# Autodesk Inventor assembly: Сборка сортировщика
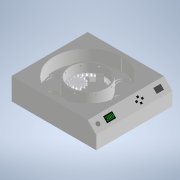
[picture p0: Inventor's stored thumbnail of the model, 180x180]
Saved by Autodesk Inventor 2022 (Build 260153000, 153)
## iProperties
Created: 2022-06-19
Part Number: Сборка сортировщика
Document SubType Name: Assembly
Designer: Admin
Author: Admin
## Documents named in this file (16)
- C:\Users\aleks\OneDrive\Рабочий стол\Проект хроматографического сборщика\Сборка сортировщика.iam
- C:\Users\aleks\OneDrive\Рабочий стол\Проект хроматографического сборщика\Барабан.ipt
- C:\Users\aleks\OneDrive\Рабочий стол\Проект хроматографического сборщика\Корпус.ipt
- C:\Users\aleks\OneDrive\Рабочий стол\Проект хроматографического сборщика\короб для подшипника.ipt
- C:\Users\aleks\OneDrive\Рабочий стол\Проект хроматографического сборщика\штырёк.ipt
- C:\Users\aleks\OneDrive\Рабочий стол\Проект хроматографического сборщика\Подшипник.ipt
- C:\Users\aleks\OneDrive\Рабочий стол\Проект хроматографического сборщика\Шаговик.ipt
- C:\Users\aleks\OneDrive\Рабочий стол\Старый сортировщик\Хромотаграфический сборщик модель\Детали\Вал.ipt
- C:\Users\aleks\OneDrive\Рабочий стол\Проект хроматографического сборщика\Healical Gear (12R@30.00 m=3.0).ipt
- C:\Users\aleks\OneDrive\Рабочий стол\Проект хроматографического сборщика\Healical Gear (32R@30.00 m=3.0).ipt
- C:\Users\aleks\OneDrive\Рабочий стол\Проект хроматографического сборщика\Держатель лазера.ipt
- C:\Users\aleks\OneDrive\Рабочий стол\Проект хроматографического сборщика\Лазер.ipt
- C:\Users\aleks\OneDrive\Рабочий стол\Проект хроматографического сборщика\Дисплей.ipt
- C:\Users\aleks\OneDrive\Рабочий стол\Проект хроматографического сборщика\Кнопки на плате.iam
- C:\Users\aleks\OneDrive\Рабочий стол\Проект хроматографического сборщика\Кнопка.ipt
- C:\Users\aleks\OneDrive\Рабочий стол\Проект хроматографического сборщика\Измеритель заряда.ipt
## Components (24 placed, 15 different names)
1. Барабан:1 — Заподлицо:1, Заподлицо:2, Заподлицо:3, Заподлицо:4, Совмещение:1, Совмещение:2, Совмещение:3, Совмещение:4, Совмещение:5, Совмещение:6, Совмещение:7, Совмещение:8, Заподлицо:5, Совмещение:9, Совмещение:15, ЗубчПер:2
2. Корпус:1 — Заподлицо:5, Совмещение:9, Совмещение:10, Совмещение:11, Совмещение:12, Совмещение:16, Совмещение:17, Совмещение:18, Совмещение:20, Совмещение:21, Заподлицо:8, Совмещение:22, Совмещение:23, Заподлицо:9, Совмещение:24, Совмещение:25, Совмещение:26, Совмещение:27, Совмещение:28
3. короб для подшипника:1 — Жесткий:2, Заподлицо:4, Совмещение:7, Совмещение:8
4. короб для подшипника:2 — Жесткий:1, Заподлицо:1, Совмещение:1, Совмещение:2
5. короб для подшипника:3 — Жесткий:3, Заподлицо:2, Совмещение:5, Совмещение:6
6. короб для подшипника:4 — Жесткий:4, Заподлицо:3, Совмещение:3, Совмещение:4
7. штырёк:2 — С поворотом:1, Жесткий:1
8. штырёк:3 — С поворотом:3, Жесткий:3
9. штырёк:4 — С поворотом:4, Жесткий:4
10. штырёк:5 — С поворотом:2, Жесткий:2
11. Подшипник:1 — С поворотом:1
12. Подшипник:2 — С поворотом:2
13. Подшипник:3 — С поворотом:3
14. Подшипник:4 — С поворотом:4
15. Шаговик:1 — Совмещение:10, Совмещение:11, Совмещение:12, Совмещение:13, Совмещение:14
16. Вал:1 — Совмещение:13, Совмещение:14, С поворотом:5
17. Healical Gear (12R@30.00 m=3.0):1 — С поворотом:5, Заподлицо:6, ЗубчПер:1
18. Healical Gear (32R@30.00 m=3.0):1 — Совмещение:15, Заподлицо:6, ЗубчПер:1, ЗубчПер:2
19. Держатель лазера:1 — Совмещение:16, Совмещение:17, Совмещение:18, Совмещение:19, Заподлицо:7
20. Лазер:1 — Совмещение:19, Заподлицо:7
21. Дисплей:1 — Заподлицо:9, Совмещение:24, Совмещение:25
22. Кнопки на плате:1 [sub-assembly] — Совмещение:26, Совмещение:27, Совмещение:28
23. Кнопка:1 — Совмещение:20, Совмещение:21
24. Измеритель заряда:1 — Заподлицо:8, Совмещение:22, Совмещение:23
## Relationships (48: Mate 28, Flush 9, RevoluteJoint 5, WeldJoint 4, RelateRotation 2)
- С поворотом:1 [RevoluteJoint]: штырёк:2 ↔ Подшипник:1
- С поворотом:2 [RevoluteJoint]: штырёк:5 ↔ Подшипник:2
- С поворотом:3 [RevoluteJoint]: штырёк:3 ↔ Подшипник:3
- С поворотом:4 [RevoluteJoint]: штырёк:4 ↔ Подшипник:4
- Жесткий:1 [WeldJoint]: короб для подшипника:2 ↔ штырёк:2
- Жесткий:2 [WeldJoint]: короб для подшипника:1 ↔ штырёк:5
- Жесткий:3 [WeldJoint]: короб для подшипника:3 ↔ штырёк:3
- Жесткий:4 [WeldJoint]: короб для подшипника:4 ↔ штырёк:4
- Заподлицо:1 [Flush]: Барабан:1 ↔ короб для подшипника:2
- Заподлицо:2 [Flush]: Барабан:1 ↔ короб для подшипника:3
- Заподлицо:3 [Flush]: Барабан:1 ↔ короб для подшипника:4
- Заподлицо:4 [Flush]: Барабан:1 ↔ короб для подшипника:1
- Совмещение:1 [Mate] (0.1 mm): Барабан:1 ↔ короб для подшипника:2
- Совмещение:2 [Mate] (0.1 mm): Барабан:1 ↔ короб для подшипника:2
- Совмещение:3 [Mate] (0.1 mm): Барабан:1 ↔ короб для подшипника:4
- Совмещение:4 [Mate] (0.1 mm): Барабан:1 ↔ короб для подшипника:4
- Совмещение:5 [Mate] (0.1 mm): Барабан:1 ↔ короб для подшипника:3
- Совмещение:6 [Mate] (0.1 mm): Барабан:1 ↔ короб для подшипника:3
- Совмещение:7 [Mate]: Барабан:1 ↔ короб для подшипника:1
- Совмещение:8 [Mate]: Барабан:1 ↔ короб для подшипника:1
- Заподлицо:5 [Flush] (-20.359 mm): Барабан:1 ↔ Корпус:1
- Совмещение:9 [Mate]: Барабан:1 ↔ Корпус:1
- Совмещение:10 [Mate]: Корпус:1 ↔ Шаговик:1
- Совмещение:11 [Mate]: Корпус:1 ↔ Шаговик:1
- Совмещение:12 [Mate]: Корпус:1 ↔ Шаговик:1
- Совмещение:13 [Mate]: Шаговик:1 ↔ Вал:1
- Совмещение:14 [Mate]: Шаговик:1 ↔ Вал:1
- С поворотом:5 [RevoluteJoint]: Вал:1 ↔ Healical Gear (12R@30.00 m=3.0):1
- Совмещение:15 [Mate]: Барабан:1 ↔ Healical Gear (32R@30.00 m=3.0):1
- Заподлицо:6 [Flush]: Healical Gear (12R@30.00 m=3.0):1 ↔ Healical Gear (32R@30.00 m=3.0):1
- ЗубчПер:1 [RelateRotation] (0.375 ul): Healical Gear (12R@30.00 m=3.0):1 ↔ Healical Gear (32R@30.00 m=3.0):1
- Совмещение:16 [Mate]: Корпус:1 ↔ Держатель лазера:1
- Совмещение:17 [Mate]: Корпус:1 ↔ Держатель лазера:1
- Совмещение:18 [Mate]: Корпус:1 ↔ Держатель лазера:1
- Совмещение:19 [Mate]: Держатель лазера:1 ↔ Лазер:1
- Заподлицо:7 [Flush]: Держатель лазера:1 ↔ Лазер:1
- ЗубчПер:2 [RelateRotation] (1 ul): Барабан:1 ↔ Healical Gear (32R@30.00 m=3.0):1
- Совмещение:20 [Mate]: Корпус:1 ↔ Кнопка:1
- Совмещение:21 [Mate]: Корпус:1 ↔ Кнопка:1
- Заподлицо:8 [Flush]: Корпус:1 ↔ Измеритель заряда:1
- Совмещение:22 [Mate]: Корпус:1 ↔ Измеритель заряда:1
- Совмещение:23 [Mate]: Корпус:1 ↔ Измеритель заряда:1
- Заподлицо:9 [Flush]: Корпус:1 ↔ Дисплей:1
- Совмещение:24 [Mate]: Корпус:1 ↔ Дисплей:1
- Совмещение:25 [Mate]: Корпус:1 ↔ Дисплей:1
- Совмещение:26 [Mate]: Корпус:1 ↔ Кнопки на плате:1
- Совмещение:27 [Mate]: Корпус:1 ↔ Кнопки на плате:1
- Совмещение:28 [Mate]: Корпус:1 ↔ Кнопки на плате:1
